# Autodesk Inventor assembly: jetracer
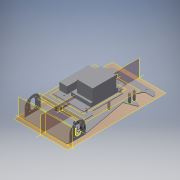
[picture p0: Inventor's stored thumbnail of the model, 180x180]
Saved by Autodesk Inventor 2019 (Build 230136000, 136)
## iProperties
Created: 2021-05-27
Part Number: jetracer
Material: Generisch
Document SubType Name: Assembly
Designer: Lukas
Author: Lukas
## Documents named in this file (6)
- C:\Users\Lukas\OneDrive\Studium 5. Sem\FachPro\jetracer.iam
- C:\Users\Lukas\OneDrive\Studium 5. Sem\FachPro\grundplatte.ipt
- C:\Users\Lukas\OneDrive\Studium 5. Sem\FachPro\waveshare_expansion_board.ipt
- C:\Users\Lukas\OneDrive\Studium 5. Sem\FachPro\abstandshalter_26mm.ipt
- C:\Users\Lukas\OneDrive\Studium 5. Sem\FachPro\abstandshalter_22mm.ipt
- C:\Users\Lukas\OneDrive\Studium 5. Sem\FachPro\jetson.ipt
## Components (11 placed, 5 different names)
1. grundplatte:1 — Passend:1, Passend:2, Einfügen:1, Einfügen:2, Einfügen:3, Einfügen:4, Einfügen:5, Einfügen:6, Einfügen:7, Einfügen:8, Einfügen:9, Einfügen:10, Passend:3, Passend:4
2. waveshare_expansion_board:1 — Passend:2, Einfügen:1, Einfügen:2, Einfügen:11, Einfügen:12
3. abstandshalter_26mm:1 — Einfügen:6
4. abstandshalter_26mm:2 — Einfügen:3
5. abstandshalter_26mm:3 — Einfügen:5
6. abstandshalter_26mm:4 — Einfügen:4
7. abstandshalter_22mm:1 — Einfügen:10
8. abstandshalter_22mm:2 — Einfügen:9
9. abstandshalter_22mm:3 — Einfügen:7
10. abstandshalter_22mm:4 — Einfügen:8
11. jetson:1 — Einfügen:11, Einfügen:12
## Relationships (16: Insert 12, Mate 4)
- Passend:1 [Mate]: grundplatte:1
- Passend:2 [Mate] (26 mm): grundplatte:1 ↔ waveshare_expansion_board:1
- Einfügen:1 [Insert] (26 mm): grundplatte:1 ↔ waveshare_expansion_board:1
- Einfügen:2 [Insert] (26 mm): grundplatte:1 ↔ waveshare_expansion_board:1
- Einfügen:3 [Insert]: grundplatte:1 ↔ abstandshalter_26mm:2
- Einfügen:4 [Insert]: grundplatte:1 ↔ abstandshalter_26mm:4
- Einfügen:5 [Insert]: grundplatte:1 ↔ abstandshalter_26mm:3
- Einfügen:6 [Insert]: grundplatte:1 ↔ abstandshalter_26mm:1
- Einfügen:7 [Insert]: grundplatte:1 ↔ abstandshalter_22mm:3
- Einfügen:8 [Insert]: grundplatte:1 ↔ abstandshalter_22mm:4
- Einfügen:9 [Insert]: grundplatte:1 ↔ abstandshalter_22mm:2
- Einfügen:10 [Insert]: grundplatte:1 ↔ abstandshalter_22mm:1
- Einfügen:11 [Insert]: waveshare_expansion_board:1 ↔ jetson:1
- Passend:3 [Mate]: grundplatte:1
- Passend:4 [Mate]: grundplatte:1
- Einfügen:12 [Insert]: waveshare_expansion_board:1 ↔ jetson:1
